# Autodesk Inventor assembly: HarmonicDrive
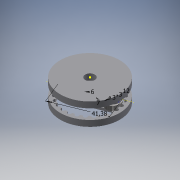
[picture p0: Inventor's stored thumbnail of the model, 180x180]
Saved by Autodesk Inventor 2018.3 (Build 223284000, 284)
## iProperties
Created: 2018-06-22
Part Number: HarmonicDrive
Material: Generisch
Document SubType Name: Assembly
Designer: JochenAlt
Author: JochenAlt
## Documents named in this file (6)
- D:\Projects\Omniwheel\HarmonicDrive.iam
- D:\Projects\Omniwheel\HarmonicDrive.ipt
- D:\Projects\Omniwheel\HarmonicDrive-WaveGenerator.ipt
- D:\Projects\Omniwheel\CircularSpline.ipt
- C:\Users\JochenAlt\Documents\Inventor\Content Center Files\R2018\de-DE\SKF - Single row ball bearings\SKF604.ipt
- D:\Projects\Omniwheel\HarmonicDrive-WaveGenerator-Bottom.ipt
## Components (6 placed, 5 different names)
1. Harmonic Drive:1 — Passend:3, Passend:5
2. HarmonicDrive-WaveGenerator:1 — Passend:3, Passend:4, Passend:10, Passend:11
3. CircularSpline:1
4. SKF- Kugellager, einreihig SKF604:2 — Passend:8, Passend:9, Passend:10
5. SKF- Kugellager, einreihig SKF604:1 — Passend:4, Passend:6, Passend:7
6. HarmonicDrive-WaveGenerator-Bottom:1 — Passend:5, Passend:6, Passend:7, Passend:8, Passend:9, Passend:11
## Relationships (9: Mate 9)
- Passend:3 [Mate]: Harmonic Drive:1 ↔ HarmonicDrive-WaveGenerator:1
- Passend:4 [Mate]: HarmonicDrive-WaveGenerator:1 ↔ SKF- Kugellager, einreihig SKF604:1
- Passend:5 [Mate]: Harmonic Drive:1 ↔ HarmonicDrive-WaveGenerator-Bottom:1
- Passend:6 [Mate]: SKF- Kugellager, einreihig SKF604:1 ↔ HarmonicDrive-WaveGenerator-Bottom:1
- Passend:7 [Mate]: SKF- Kugellager, einreihig SKF604:1 ↔ HarmonicDrive-WaveGenerator-Bottom:1
- Passend:8 [Mate]: SKF- Kugellager, einreihig SKF604:2 ↔ HarmonicDrive-WaveGenerator-Bottom:1
- Passend:9 [Mate]: SKF- Kugellager, einreihig SKF604:2 ↔ HarmonicDrive-WaveGenerator-Bottom:1
- Passend:10 [Mate]: HarmonicDrive-WaveGenerator:1 ↔ SKF- Kugellager, einreihig SKF604:2
- Passend:11 [Mate]: HarmonicDrive-WaveGenerator:1 ↔ HarmonicDrive-WaveGenerator-Bottom:1
